# Autodesk Inventor assembly: Kołnierz z siłownikiem
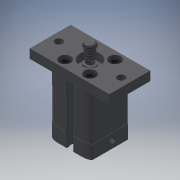
[picture p0: Inventor's stored thumbnail of the model, 180x180]
Saved by Autodesk Inventor 2017 (Build 210142000, 142)
## iProperties
Created: 2018-05-29
Part Number: Kołnierz z siłownikiem
Document SubType Name: Assembly
Designer: Pies
Author: Pies
## Documents named in this file (3)
- C:\Users\Pies\Desktop\Rzeczy\AGH\Semestr 2\ZIPK\Chwytak\Moj_Chwd_Pytak\Inventorowe chwytaki\Kołnierz z siłownikiem.iam
- C:\Users\Pies\Desktop\Rzeczy\AGH\Semestr 2\ZIPK\Chwytak\Moj_Chwd_Pytak\Inventorowe chwytaki\Kołnierz\537247 FNC-20.iam
- C:\Users\Pies\Desktop\Rzeczy\AGH\Semestr 2\ZIPK\Chwytak\Moj_Chwd_Pytak\Inventorowe chwytaki\Silownik\536236 ADN-20-15-A-P-A---(asm_0).iam
## Components (2 placed, 2 different names)
1. 537247 FNC-20:1 [sub-assembly] — Rigid:1
2. 536236 ADN-20-15-A-P-A---(asm_0):1 [sub-assembly] — Rigid:1
## Relationships (1: WeldJoint 1)
- Rigid:1 [WeldJoint]: 537247 FNC-20:1 ↔ 536236 ADN-20-15-A-P-A---(asm_0):1
